# Autodesk Inventor assembly: 1410 LaserShow
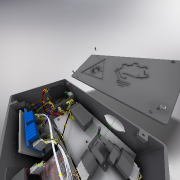
[picture p0: Inventor's stored thumbnail of the model, 180x180]
Saved by Autodesk Inventor 2017 (Build 210142000, 142)
## iProperties
Part Number: 1410 LaserShow
Material: Générique
Document SubType Name: Assembly
Designer: Adrien MARY
Stock Number: 1410-00-00
Project: 1410 LaserShow
Author: Adrien MARY
## Documents named in this file (18)
- W:\Professionnel\Conception FABLAB\1410-LaserShow\1410 LaserShow.iam
- W:\Professionnel\Conception FABLAB\1410-LaserShow\1410-01 Boitier\1410-01-01 Partie inferieur.ipt
- W:\Professionnel\Conception FABLAB\1410-LaserShow\1410-02 Moteur + laser\1410-02-00 Moteur + Laser.iam
- W:\Professionnel\Conception FABLAB\1410-LaserShow\1410-03 Composant electronique\1410-03-06 Plug+prise.ipt
- W:\Professionnel\Conception FABLAB\1410-LaserShow\1410-03 Composant electronique\1410-03-03 Ecran.ipt
- W:\Professionnel\Conception FABLAB\1410-LaserShow\1410-03 Composant electronique\1410-03-02 Carte electronique alimentation.ipt
- W:\Professionnel\Conception FABLAB\1410-LaserShow\1410-03 Composant electronique\1410-03-07 Carte electronique moteur.ipt
- W:\Professionnel\Conception FABLAB\1410-LaserShow\1410-03 Composant electronique\1410-03-01 Carte electronique laser.ipt
- W:\Professionnel\Conception FABLAB\1410-LaserShow\1410-03 Composant electronique\1410-03-04 Potentiomètre.ipt
- W:\Professionnel\Conception FABLAB\1410-LaserShow\1410-03 Composant electronique\1410-03-05 Ventillateur_60x60x11.ipt
- W:\Professionnel\Conception FABLAB\1410-LaserShow\1410-90 Centre de contenu\fr-FR\ISO 7049 - C-H(2)\ISO 7049 - ST 3,5 x 13 - C - H.ipt
- W:\Professionnel\Conception FABLAB\1410-LaserShow\1410-90 Centre de contenu\fr-FR\ISO 7046-1 H(1)\ISO 7046-1 - M3 x 8 - 4.8 - H - ISO.ipt
- W:\Professionnel\Conception FABLAB\1410-LaserShow\1410-90 Centre de contenu\fr-FR\ISO 4762(2)\ISO 4762 - M3 x 16ISO.ipt
- W:\Professionnel\Conception FABLAB\1410-LaserShow\1410-90 Centre de contenu\fr-FR\ISO 4032(2)\ISO 4032 - M3 - ISO.ipt
- W:\Professionnel\Conception FABLAB\1410-LaserShow\1410-01 Boitier\1410-01-02 Couvercle.ipt
- W:\Professionnel\Conception FABLAB\1410-LaserShow\1410-90 Centre de contenu\fr-FR\ISO 4762(2)\ISO 4762 - M3 x 8ISO.ipt
- W:\Professionnel\Conception FABLAB\1410-LaserShow\1410-01 Boitier\1410-01-05 Capuchon.ipt
- W:\Professionnel\Conception FABLAB\1410-LaserShow\1410-50 Cable et faisceau\1410-50 Cable et faisceau.iam
## Components (44 placed, 17 different names)
1. 1410-50 Cable et faisceau [sub-assembly]
2. 1410-01-05 Capuchon:1 — Logement:41, Angle:2
3. ISO 4762 M3 x 8:4 — Logement:39
4. ISO 4762 M3 x 8:3 — Ouverture vis
5. ISO 4762 M3 x 8:2 — Logement:38
6. ISO 4762 M3 x 8:1 — Logement:40
7. 1410-01-02 Couvercle:1 — Ouverture vis, Logement:38, Logement:39, Logement:40, Angle:3, Affleurement:1, Placage:11
8. 1410-01-01 Partie inferieur:1 — Logement:1, Logement:2, Logement:3, Placage:1, Logement:4, Placage:2, Placage:3, Logement:5, Placage:4, Placage:5, Placage:6, Logement:6, Placage:7, Angle:1, Placage:8, Placage:9, Logement:7, Placage:10, Logement:25, Logement:26, Logement:27, Logement:28, Logement:33, Logement:34, Logement:35, Logement:36, Logement:41, Placage:11
9. ISO 7049 - C-H ST 3,5 x 13 - C - H:8 — Logement:14
10. ISO 7049 - C-H ST 3,5 x 13 - C - H:7 — Logement:15
11. ISO 7049 - C-H ST 3,5 x 13 - C - H:6 — Logement:13
12. ISO 7049 - C-H ST 3,5 x 13 - C - H:5 — Logement:12
13. 1410-02-00 Moteur + Laser:1 [sub-assembly] — Logement:1, Logement:2, Logement:12, Logement:13, Logement:14, Logement:15
14. ISO 7049 - C-H ST 3,5 x 13 - C - H:11 — Logement:19
15. ISO 7049 - C-H ST 3,5 x 13 - C - H:12 — Logement:20
16. 1410-03-01 Carte electronique laser:1 — Logement:6, Placage:7, Logement:19, Logement:20
17. 1410-03-02 Carte electronique alimentation:1 — Placage:3, Logement:5, Logement:8, Logement:9, Logement:10, Logement:18
18. ISO 7049 - C-H ST 3,5 x 13 - C - H:1 — Logement:8
19. ISO 7049 - C-H ST 3,5 x 13 - C - H:2 — Logement:10
20. ISO 7049 - C-H ST 3,5 x 13 - C - H:3 — Logement:9
21. ISO 7049 - C-H ST 3,5 x 13 - C - H:4 — Logement:18
22. ISO 7046-1 H M3 x 8 - 4.8 - H:1 — Logement:21
23. ISO 7046-1 H M3 x 8 - 4.8 - H:2 — Logement:22
24. ISO 4032 M3:6
25. ISO 4032 M3:5
26. 1410-03-06 Plug+prise:1 — Logement:3, Placage:1, Logement:21, Logement:22
27. 1410-03-04 Potentiomètre:1 — Angle:1, Placage:8, Placage:9
28. 1410-03-03 Ecran:1 — Logement:4, Placage:2
29. ISO 7049 - C-H ST 3,5 x 13 - C - H:9 — Logement:17
30. ISO 7049 - C-H ST 3,5 x 13 - C - H:10 — Logement:16
31. 1410-03-07 Carte electronique moteur:1 — Placage:4, Placage:5, Placage:6, Logement:16, Logement:17
32. ISO 4762 M3 x 16:1 — Logement:25
33. ISO 4762 M3 x 16:2 — Logement:26
34. ISO 4762 M3 x 16:3 — Logement:27
35. ISO 4762 M3 x 16:4 — Logement:28
36. ISO 4032 M3:1
37. ISO 4032 M3:2
38. ISO 4032 M3:3
39. ISO 4032 M3:4
40. 1410-03-05 Ventillateur_60x60x11:1 — Logement:7, Placage:10
41. ISO 4032 M3:7 — Logement:33
42. ISO 4032 M3:8 — Logement:34
43. ISO 4032 M3:9 — Logement:36
44. ISO 4032 M3:10 — Logement:35
## Relationships (55: Insert 40, Mate 11, Angle 3, Flush 1)
- Logement:1 [Insert]: 1410-01-01 Partie inferieur:1 ↔ 1410-02-00 Moteur + Laser:1
- Logement:2 [Insert]: 1410-01-01 Partie inferieur:1 ↔ 1410-02-00 Moteur + Laser:1
- Logement:3 [Insert]: 1410-01-01 Partie inferieur:1 ↔ 1410-03-06 Plug+prise:1
- Placage:1 [Mate]: 1410-01-01 Partie inferieur:1 ↔ 1410-03-06 Plug+prise:1
- Logement:4 [Insert]: 1410-01-01 Partie inferieur:1 ↔ 1410-03-03 Ecran:1
- Placage:2 [Mate]: 1410-01-01 Partie inferieur:1 ↔ 1410-03-03 Ecran:1
- Placage:3 [Mate]: 1410-01-01 Partie inferieur:1 ↔ 1410-03-02 Carte electronique alimentation:1
- Logement:5 [Insert]: 1410-01-01 Partie inferieur:1 ↔ 1410-03-02 Carte electronique alimentation:1
- Placage:4 [Mate]: 1410-01-01 Partie inferieur:1 ↔ 1410-03-07 Carte electronique moteur:1
- Placage:5 [Mate]: 1410-01-01 Partie inferieur:1 ↔ 1410-03-07 Carte electronique moteur:1
- Placage:6 [Mate]: 1410-01-01 Partie inferieur:1 ↔ 1410-03-07 Carte electronique moteur:1
- Logement:6 [Insert]: 1410-01-01 Partie inferieur:1 ↔ 1410-03-01 Carte electronique laser:1
- Placage:7 [Mate]: 1410-01-01 Partie inferieur:1 ↔ 1410-03-01 Carte electronique laser:1
- Angle:1 (180 deg): 1410-01-01 Partie inferieur:1 ↔ 1410-03-04 Potentiomètre:1
- Placage:8 [Mate]: 1410-01-01 Partie inferieur:1 ↔ 1410-03-04 Potentiomètre:1
- Placage:9 [Mate]: 1410-01-01 Partie inferieur:1 ↔ 1410-03-04 Potentiomètre:1
- Logement:7 [Insert]: 1410-01-01 Partie inferieur:1 ↔ 1410-03-05 Ventillateur_60x60x11:1
- Placage:10 [Mate]: 1410-01-01 Partie inferieur:1 ↔ 1410-03-05 Ventillateur_60x60x11:1
- Logement:8 [Insert]: 1410-03-02 Carte electronique alimentation:1 ↔ ISO 7049 - C-H ST 3,5 x 13 - C - H:1
- Logement:9 [Insert]: 1410-03-02 Carte electronique alimentation:1 ↔ ISO 7049 - C-H ST 3,5 x 13 - C - H:3
- Logement:10 [Insert]: 1410-03-02 Carte electronique alimentation:1 ↔ ISO 7049 - C-H ST 3,5 x 13 - C - H:2
- Logement:12 [Insert]: ISO 7049 - C-H ST 3,5 x 13 - C - H:5 ↔ 1410-02-00 Moteur + Laser:1
- Logement:13 [Insert]: ISO 7049 - C-H ST 3,5 x 13 - C - H:6 ↔ 1410-02-00 Moteur + Laser:1
- Logement:14 [Insert]: ISO 7049 - C-H ST 3,5 x 13 - C - H:8 ↔ 1410-02-00 Moteur + Laser:1
- Logement:15 [Insert]: ISO 7049 - C-H ST 3,5 x 13 - C - H:7 ↔ 1410-02-00 Moteur + Laser:1
- Logement:16 [Insert]: ISO 7049 - C-H ST 3,5 x 13 - C - H:10 ↔ 1410-03-07 Carte electronique moteur:1
- Logement:17 [Insert]: ISO 7049 - C-H ST 3,5 x 13 - C - H:9 ↔ 1410-03-07 Carte electronique moteur:1
- Logement:18 [Insert]: 1410-03-02 Carte electronique alimentation:1 ↔ ISO 7049 - C-H ST 3,5 x 13 - C - H:4
- Logement:19 [Insert]: ISO 7049 - C-H ST 3,5 x 13 - C - H:11 ↔ 1410-03-01 Carte electronique laser:1
- Logement:20 [Insert]: ISO 7049 - C-H ST 3,5 x 13 - C - H:12 ↔ 1410-03-01 Carte electronique laser:1
- Logement:21 [Insert]: ISO 7046-1 H M3 x 8 - 4.8 - H:1 ↔ 1410-03-06 Plug+prise:1
- Logement:22 [Insert]: ISO 7046-1 H M3 x 8 - 4.8 - H:2 ↔ 1410-03-06 Plug+prise:1
- [Insert]: 1410-01-01 Partie inferieur:1 ↔ ISO 4032 M3:6
- [Insert]: 1410-01-01 Partie inferieur:1 ↔ ISO 4032 M3:5
- Logement:25 [Insert]: 1410-01-01 Partie inferieur:1 ↔ ISO 4762 M3 x 16:1
- Logement:26 [Insert]: 1410-01-01 Partie inferieur:1 ↔ ISO 4762 M3 x 16:2
- Logement:27 [Insert]: 1410-01-01 Partie inferieur:1 ↔ ISO 4762 M3 x 16:3
- Logement:28 [Insert]: 1410-01-01 Partie inferieur:1 ↔ ISO 4762 M3 x 16:4
- [Insert]: ISO 4032 M3:2 ↔ 1410-03-05 Ventillateur_60x60x11:1
- [Insert]: ISO 4032 M3:4 ↔ 1410-03-05 Ventillateur_60x60x11:1
- [Insert]: ISO 4032 M3:3 ↔ 1410-03-05 Ventillateur_60x60x11:1
- [Insert]: ISO 4032 M3:1 ↔ 1410-03-05 Ventillateur_60x60x11:1
- Logement:33 [Insert]: 1410-01-01 Partie inferieur:1 ↔ ISO 4032 M3:7
- Logement:34 [Insert]: 1410-01-01 Partie inferieur:1 ↔ ISO 4032 M3:8
- Logement:35 [Insert]: 1410-01-01 Partie inferieur:1 ↔ ISO 4032 M3:10
- Logement:36 [Insert]: 1410-01-01 Partie inferieur:1 ↔ ISO 4032 M3:9
- Ouverture vis [Insert] (35 mm): ISO 4762 M3 x 8:3 ↔ 1410-01-02 Couvercle:1
- Logement:38 [Insert] (35 mm): ISO 4762 M3 x 8:2 ↔ 1410-01-02 Couvercle:1
- Logement:39 [Insert] (35 mm): ISO 4762 M3 x 8:4 ↔ 1410-01-02 Couvercle:1
- Logement:40 [Insert] (35 mm): ISO 4762 M3 x 8:1 ↔ 1410-01-02 Couvercle:1
- Logement:41 [Insert]: 1410-01-05 Capuchon:1 ↔ 1410-01-01 Partie inferieur:1
- Angle:2 (0 deg): 1410-01-05 Capuchon:1
- Angle:3 (-30 deg): 1410-01-02 Couvercle:1
- Affleurement:1 [Flush]: 1410-01-02 Couvercle:1
- Placage:11 [Mate]: 1410-01-02 Couvercle:1 ↔ 1410-01-01 Partie inferieur:1
## Named parameters: Ouyverture_vis = 35 mm
